# Autodesk Inventor assembly: LETU-Maker_Base_LM3032
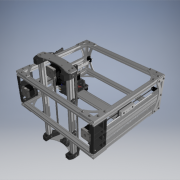
[picture p0: Inventor's stored thumbnail of the model, 180x180]
Saved by Autodesk Inventor 2020.2 (Build 242310000, 310)
## iProperties
Created: 2020-04-07
Part Number: LETU-Maker_Base_LM3032
Document SubType Name: Assembly
Designer: rah75
Author: rah75
## Documents named in this file (5)
- C:\Users\rah75\Documents\GitHub\LETU-Maker\CAD\Autodesk Inventor\Base_3001-5999\Assemblies\LETU-Maker_Base_LM3032.iam
- C:\Users\rah75\Documents\GitHub\LETU-Maker\CAD\Autodesk Inventor\Base_3001-5999\Frame\Assemblies\Frame_LM3030.iam
- C:\Users\rah75\Documents\GitHub\LETU-Maker\CAD\Autodesk Inventor\Base_3001-5999\X-Axis\Assemblies\X-Axis_LM3006.iam
- C:\Users\rah75\Documents\GitHub\LETU-Maker\CAD\Autodesk Inventor\Base_3001-5999\Y-Axis\Assemblies\Y_Axis_LM3021.iam
- C:\Users\rah75\Documents\GitHub\LETU-Maker\CAD\Autodesk Inventor\Modules_6001-9999\Extruder\Assemblies\Extruder_LM6012.iam
## Components (4 placed, 4 different names)
1. Frame_LM3030:1 [sub-assembly] — Mate:1, Mate:2, Mate:3, Mate:4, Mate:5
2. X-Axis_LM3006:1 [sub-assembly] — Mate:1, Mate:2, Insert:1, Mate:6
3. Y_Axis_LM3021:1 [sub-assembly] — Mate:3, Mate:4, Mate:5
4. Extruder_LM6012:1 [sub-assembly] — Insert:1, Mate:6
## Relationships (7: Mate 6, Insert 1)
- Mate:1: Frame_LM3030:1 ↔ X-Axis_LM3006:1
- Mate:2: Frame_LM3030:1 ↔ X-Axis_LM3006:1
- Mate:3: Frame_LM3030:1 ↔ Y_Axis_LM3021:1
- Mate:4: Frame_LM3030:1 ↔ Y_Axis_LM3021:1
- Mate:5 (112.5 mm): Frame_LM3030:1 ↔ Y_Axis_LM3021:1
- Insert:1: X-Axis_LM3006:1 ↔ Extruder_LM6012:1
- Mate:6: X-Axis_LM3006:1 ↔ Extruder_LM6012:1
